# Autodesk Inventor assembly: ЛЦМК.30000.30.00.00 СБ Крепление
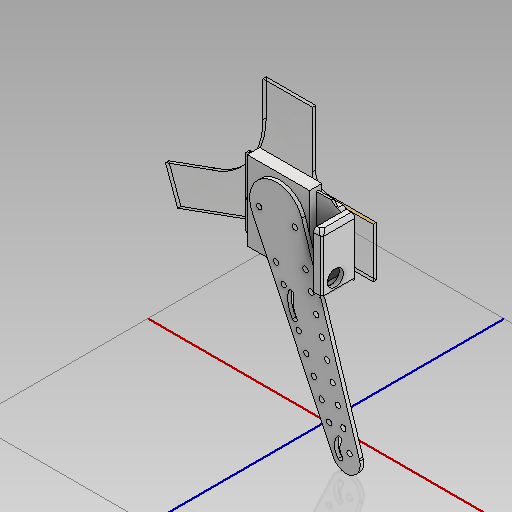
[picture p0: Inventor's stored thumbnail of the model, 512x512]
Saved by Autodesk Inventor 2021.2 (Build 252289000, 289)
## iProperties
Created: 2025-11-22
Part Number: ЛЦМК.30000.30.00.00 СБ Крепление
Document SubType Name: Assembly
Designer: Захаров
Author: Захаров
## Documents named in this file (5)
- C:\Users\User\Documents\CaseARHead1\ЛЦМК.30000.30.00.00 Крепление\ЛЦМК.30000.30.00.00 СБ Крепление.iam
- C:\Users\User\Documents\CaseARHead1\ЛЦМК.30000.30.00.00 Крепление\ЛЦМК.30000.30.00.01 Слайдер.ipt
- C:\Users\User\Documents\CaseARHead1\ЛЦМК.30000.30.00.00 Крепление\ЛЦМК.30000.30.00.02 Штанга.ipt
- C:\Users\User\Documents\CaseARHead1\ЛЦМК.30000.30.00.00 Крепление\Присоединительная часть.ipt
- C:\Users\User\Documents\CaseARHead1\ЛЦМК.30000.30.00.00 Крепление\Обхват головы.ipt
## Components (4 placed, 4 different names)
1. ЛЦМК.30000.30.00.01 Слайдер:1 — Вставка:1, Вставка:2, Совмещение:1, Заподлицо:1, Совмещение:2
2. ЛЦМК.30000.30.00.02 Штанга:1 — Вставка:1, Вставка:2
3. Присоединительная часть:1 — Совмещение:1, Заподлицо:1, Совмещение:2, Вставка:3, Вставка:4
4. Обхват головы:1 — Вставка:3, Вставка:4
## Relationships (7: Insert 4, Mate 2, Flush 1)
- Вставка:1 [Insert]: ЛЦМК.30000.30.00.01 Слайдер:1 ↔ ЛЦМК.30000.30.00.02 Штанга:1
- Вставка:2 [Insert]: ЛЦМК.30000.30.00.01 Слайдер:1 ↔ ЛЦМК.30000.30.00.02 Штанга:1
- Совмещение:1 [Mate]: ЛЦМК.30000.30.00.01 Слайдер:1 ↔ Присоединительная часть:1
- Заподлицо:1 [Flush] (-5 mm): ЛЦМК.30000.30.00.01 Слайдер:1 ↔ Присоединительная часть:1
- Совмещение:2 [Mate]: ЛЦМК.30000.30.00.01 Слайдер:1 ↔ Присоединительная часть:1
- Вставка:3 [Insert]: Присоединительная часть:1 ↔ Обхват головы:1
- Вставка:4 [Insert]: Присоединительная часть:1 ↔ Обхват головы:1
